# Autodesk Inventor assembly: bulkhead_assembly
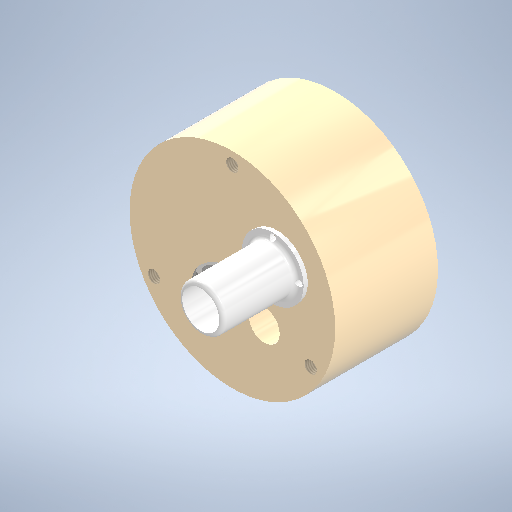
[picture p0: Inventor's stored thumbnail of the model, 512x512]
Saved by Autodesk Inventor 2025 (Build 290162010, 162A)
## iProperties
Created: 2024-07-19
Part Number: bulkhead_assembly
Document SubType Name: Assembly
Designer: HP
Author: HP
## Documents named in this file (6)
- C:\Users\HP\Desktop\Project CAD files\bulkhead_assembly.iam
- C:\Users\HP\Desktop\Project CAD files\bulkhead\bulkhead.ipt
- C:\Users\HP\Desktop\Project CAD files\charge_holder\charge_holder.ipt
- C:\Users\HP\Documents\Inventor\Content Center Files\R2025\en-US\GB 798-88\Eye bolt GB 798 M8 x 70.ipt
- C:\Users\HP\Documents\Inventor\Content Center Files\R2025\en-US\AS 1237 (2.1)\AS 1237 - 8.ipt
- C:\Users\HP\Documents\Inventor\Content Center Files\R2025\en-US\BS 3692(1)\BS 3692 - M8(1).ipt
## Components (5 placed, 5 different names)
1. bulkhead:1 — Mate:1, Mate:2, Mate:3, Insert:1, Mate:5
2. charge_holder:1 — Mate:1, Mate:2, Mate:3
3. Bolt GB/T 798-1988 M8 x 70:1 — Insert:1, Mate:4, Mate:6
4. AS 1237 (2.1) 8:1 — Mate:4, Mate:5, Mate:7
5. BS 3692 - Metric M8:1 — Mate:6, Mate:7
## Relationships (8: Mate 7, Insert 1)
- Mate:1: bulkhead:1 ↔ charge_holder:1
- Mate:2: bulkhead:1 ↔ charge_holder:1
- Mate:3: bulkhead:1 ↔ charge_holder:1
- Insert:1 (-38 mm): bulkhead:1 ↔ Bolt GB/T 798-1988 M8 x 70:1
- Mate:4: Bolt GB/T 798-1988 M8 x 70:1 ↔ AS 1237 (2.1) 8:1
- Mate:5: bulkhead:1 ↔ AS 1237 (2.1) 8:1
- Mate:6: Bolt GB/T 798-1988 M8 x 70:1 ↔ BS 3692 - Metric M8:1
- Mate:7: AS 1237 (2.1) 8:1 ↔ BS 3692 - Metric M8:1
